# Autodesk Inventor assembly: ToASI-1
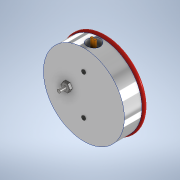
[picture p0: Inventor's stored thumbnail of the model, 180x180]
Saved by Autodesk Inventor 2020.3 (Build 243373000, 373)
## iProperties
Created: 2020-07-31
Part Number: ToASI-1
Document SubType Name: Assembly
Designer: Bruno
Author: Bruno
## Documents named in this file (6)
- C:\Users\Bruno\Desktop\Github\CAD\Inventor\For ASI\ToASI-1.iam
- C:\Users\Bruno\Desktop\Github\CAD\Inventor\Heater-Box\Box-Disk\Heater disk.ipt
- C:\Users\Bruno\Desktop\Github\CAD\Inventor\Heater-Box\Electric parts\DIN913-M5x5 socket screw flat end.ipt
- C:\Users\Bruno\Desktop\Github\CAD\Inventor\Heater-Box\Electric parts\Heater630W.ipt
- C:\Users\Bruno\Desktop\Github\CAD\Inventor\Heater-Box\Electric parts\Thermocouple.ipt
- C:\Users\Bruno\Desktop\Github\CAD\Inventor\Heater-Box\Box-Disk\Oring 2-343.ipt
## Components (6 placed, 5 different names)
1. Heater disk:1 — Cylindrical:1, Cylindrical:2, Cylindrical:3, Cylindrical:4, Cylindrical:5
2. DIN913-M5x5 socket screw flat end:1 — Cylindrical:2
3. DIN913-M5x5 socket screw flat end:2 — Cylindrical:1
4. Heater630W:1 — Cylindrical:4
5. Thermocouple:1 — Cylindrical:3
6. Oring 2-343:1 — Cylindrical:5
## Relationships (5: CylindricalJoint 5)
- Cylindrical:1: Heater disk:1 ↔ DIN913-M5x5 socket screw flat end:2
- Cylindrical:2: Heater disk:1 ↔ DIN913-M5x5 socket screw flat end:1
- Cylindrical:3: Heater disk:1 ↔ Thermocouple:1
- Cylindrical:4: Heater disk:1 ↔ Heater630W:1
- Cylindrical:5: Heater disk:1 ↔ Oring 2-343:1
